# Autodesk Inventor assembly: first_mirror
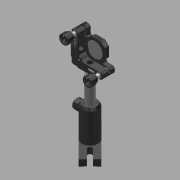
[picture p0: Inventor's stored thumbnail of the model, 180x180]
Saved by Autodesk Inventor 2018 (Build 220112000, 112)
## iProperties
Created: 2018-09-17
Part Number: first_mirror
Document SubType Name: Assembly
Designer: Robert Campbell
Author: Robert Campbell
## Documents named in this file (6)
- Y:\LaserAlignment\first_mirror.iam
- \\Mac\Home\Downloads\LaserAlignment\BA1_M-Solidworks.ipt
- \\Mac\Home\Downloads\LaserAlignment\KM100-Solidworks.ipt
- \\Mac\Home\Downloads\LaserAlignment\PF1011-F01-Solidworks.ipt
- \\Mac\Home\Downloads\LaserAlignment\PH50_M-Solidworks.ipt
- \\Mac\Home\Downloads\LaserAlignment\TR50_M-Solidworks.ipt
## Components (5 placed, 5 different names)
1. BA1_M-Solidworks:1 — Mate:3, Mate:4
2. KM100-Solidworks:1 — Mate:1, Mate:2, Mate:7, Mate:8
3. PF1011-F01-Solidworks:1 — Mate:1, Mate:2
4. PH50_M-Solidworks:1 — Mate:3, Mate:4, Mate:5, Mate:6
5. TR50_M-Solidworks:1 — Mate:5, Mate:6, Mate:7, Mate:8
## Relationships (8: Mate 8)
- Mate:1: KM100-Solidworks:1 ↔ PF1011-F01-Solidworks:1
- Mate:2: KM100-Solidworks:1 ↔ PF1011-F01-Solidworks:1
- Mate:3: BA1_M-Solidworks:1 ↔ PH50_M-Solidworks:1
- Mate:4: BA1_M-Solidworks:1 ↔ PH50_M-Solidworks:1
- Mate:5: PH50_M-Solidworks:1 ↔ TR50_M-Solidworks:1
- Mate:6 (35 mm): PH50_M-Solidworks:1 ↔ TR50_M-Solidworks:1
- Mate:7: KM100-Solidworks:1 ↔ TR50_M-Solidworks:1
- Mate:8: KM100-Solidworks:1 ↔ TR50_M-Solidworks:1
